# Autodesk Inventor assembly: Final platform assembly
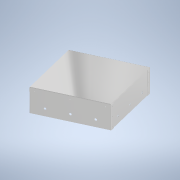
[picture p0: Inventor's stored thumbnail of the model, 180x180]
Saved by Autodesk Inventor 2020 (Build 240168000, 168)
## iProperties
Created: 2022-07-05
Part Number: Final platform assembly
Document SubType Name: Assembly
Designer: karimi2
Author: karimi2
## Documents named in this file (3)
- C:\Users\karimi2\Documents\PROJECT\src\Final platform assembly.iam
- C:\Users\karimi2\Documents\PROJECT\src\Platform Sides Assembly.iam
- C:\Users\karimi2\Documents\PROJECT\src\Platform top.ipt
## Components (2 placed, 2 different names)
1. Platform Sides Assembly:1 [sub-assembly] — Mate:1, Rigid:1
2. Platform top:1 — Mate:1, Rigid:1
## Relationships (2: Mate 1, WeldJoint 1)
- Mate:1: Platform Sides Assembly:1 ↔ Platform top:1
- Rigid:1 [WeldJoint]: Platform Sides Assembly:1 ↔ Platform top:1
